# Autodesk Inventor assembly: UntererRührer
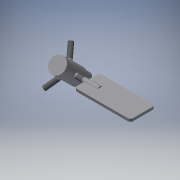
[picture p0: Inventor's stored thumbnail of the model, 180x180]
Saved by Autodesk Inventor 2017 (Build 210142000, 142)
## iProperties
Created: 2019-06-21
Part Number: UntererRührer
Document SubType Name: Assembly
Designer: Ole Simmering
Author: Ole Simmering
## Documents named in this file (3)
- C:\Users\Ole Simmering\Documents\3d modelling fun\HA5-Rührreaktor\UntererRührer.iam
- C:\Users\Ole Simmering\Documents\3d modelling fun\HA5-Rührreaktor\UntererRührer.ipt
- C:\Users\Ole Simmering\Documents\3d modelling fun\HA5-Rührreaktor\UntererRührerHalter.ipt
## Components (2 placed, 2 different names)
1. UntererRührer:1 — Insert:1
2. UntererRührerHalter:1 — Insert:1
## Relationships (1: Insert 1)
- Insert:1 (-5 mm): UntererRührer:1 ↔ UntererRührerHalter:1
